# Autodesk Inventor assembly: chassis
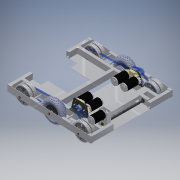
[picture p0: Inventor's stored thumbnail of the model, 180x180]
Saved by Autodesk Inventor 2016 (Build 200138000, 138)
## iProperties
Created: 2016-01-16
Part Number: chassis
Document SubType Name: Assembly
Designer: gus
Mass: 18782.9 g
Surface Area: 40799.8 cm^2
Volume: 7776.64 cm^3
Density: 2.4153 g/cm^3
Author: gus
## Documents named in this file (24)
- \\Mac\Home\Desktop\1510-stronghold-CAD-master\chassis\chassis.iam
- \\Mac\Home\Desktop\1510-stronghold-CAD-master\chassis\1x2x28.ipt
- \\Mac\Home\Desktop\1510-stronghold-CAD-master\chassis\1x2x19.ipt
- \\Mac\Home\Desktop\1510-stronghold-CAD-master\chassis\1x2x8in.ipt
- \\Mac\Home\Desktop\1510-stronghold-CAD-master\chassis\3 in churro.ipt
- \\Mac\Home\Desktop\1510-stronghold-CAD-master\chassis\side plate.ipt
- \\Mac\Home\Desktop\1510-stronghold-CAD-master\chassis\PneumaticWheel_am-0970-2.iam
- \\Mac\Home\Desktop\1510-stronghold-CAD-master\chassis\CIMple Box\CIMple Box.iam
- \\Mac\Home\Desktop\1510-stronghold-CAD-master\chassis\am-0736_S35-12DHE.ipt
- \\Mac\Home\Desktop\1510-stronghold-CAD-master\chassis\am-940a-6-HiGrip-.iam
- \\Mac\Home\Desktop\1510-stronghold-CAD-master\chassis\half-inch hex bolt.ipt
- \\Mac\Home\Desktop\1510-stronghold-CAD-master\chassis\half-inch hex nut.ipt
- \\Mac\Home\Desktop\1510-stronghold-CAD-master\chassis\wheel arm support.ipt
- \\Mac\Home\Desktop\1510-stronghold-CAD-master\roller wheels\toughbox micro\Toughbox+Nano+All+Shafts+v2-2.iam
- \\Mac\Home\Desktop\1510-stronghold-CAD-master\roller wheels\hex bearing.ipt
- \\Mac\Home\Desktop\1510-stronghold-CAD-master\chassis\chassis\Design Accelerator\Chain Drive13.iam
- \\Mac\Home\Desktop\1510-stronghold-CAD-master\chassis\chassis\Design Accelerator\Chain Drive14.iam
- \\Mac\Home\Desktop\1510-stronghold-CAD-master\chassis\chassis\Design Accelerator\Chain Drive15.iam
- \\Mac\Home\Desktop\1510-stronghold-CAD-master\chassis\chassis\Design Accelerator\Chain Drive16.iam
- \\Mac\Home\Desktop\1510-stronghold-CAD-master\chassis\chassis\Design Accelerator\Chain Drive17.iam
- \\Mac\Home\Desktop\1510-stronghold-CAD-master\chassis\skid plate.ipt
- \\Mac\Home\Desktop\1510-stronghold-CAD-master\chassis\request-piano-hinge-1\PIANO HINGE.iam
- \\Mac\Home\Desktop\1510-stronghold-CAD-master\chassis\skid plate back.ipt
- \\Mac\Home\Desktop\1510-stronghold-CAD-master\chassis\skid strip.ipt
## Components (52 placed, 19 different names)
1. 1x2x28:1 — Mate:1, Mate:2, Flush:2, Mate:4, Flush:4, Flush:6, Mate:19, Rotational:7, Rotational:8, Cylindrical:25, Rotational:18, Rotational:29, Cylindrical:22, Mate:41, Mate:57, Mate:58, Flush:49, Flush:53
2. 1x2x19:1 — Mate:1, Flush:2, Mate:12, Mate:13, Flush:22
3. 1x2x19:2 — Mate:2, Mate:34, Flush:43, Flush:44, Mate:71, Mate:72, Flush:48, Mate:73
4. 1x2x8in:1 — Mate:8, Flush:10, Mate:13, Mate:35, Flush:52
5. 1x2x8in:2 — Mate:4, Flush:4, Flush:6, Mate:9, Flush:11, Mate:12, Mate:62
6. 3 in churro:1 — Mate:10, Mate:67
7. 3 in churro:2 — Mate:11, Mate:65
8. 3 in churro:3 — Mate:36, Mate:69
9. 3 in churro:4 — Mate:37, Mate:70
10. side plate:1 — Mate:8, Flush:10, Mate:21, Rotational:23, Rotational:24, Rotational:25, Mate:61, Mate:63, Mate:68, Mate:69, Mate:70
11. side plate:2 — Mate:9, Flush:11, Mate:10, Mate:11, Mate:22, Rotational:26, Rotational:27, Rotational:28, Mate:62, Mate:64, Mate:65, Mate:66, Mate:67, Mate:77
12. PneumaticWheel_am-0970-2:1 [sub-assembly] — Rotational:20, Flush:39, Flush:40
13. 1x2x8in:3 — Mate:19, Mate:22, Mate:53, Flush:34, Flush:54, Mate:77, Flush:56
14. 1x2x8in:4 — Mate:21, Mate:33, Flush:20, Flush:21, Flush:28, Mate:39, Mate:61, Flush:56, Flush:57
15. am-0736_S35-12DHE:1 — Cylindrical:2, Mate:49
16. am-0736_S35-12DHE:2 — Mate:50, Cylindrical:26
17. am-940a-6-HiGrip-:1 [sub-assembly] — Cylindrical:25, Flush:42
18. am-940a-6-HiGrip-:2 [sub-assembly] — Cylindrical:22, Flush:41
19. am-940a-6-HiGrip-:3 [sub-assembly] — Cylindrical:23, Flush:40
20. am-940a-6-HiGrip-:4 [sub-assembly] — Cylindrical:24, Flush:39
21. half-inch hex bolt:2 — Rotational:12
22. half-inch hex bolt:4 — Rotational:14
23. half-inch hex bolt:5 — Rotational:7
24. half-inch hex bolt:6 — Rotational:8
25. PneumaticWheel_am-0970-2:2 [sub-assembly] — Rotational:29, Flush:41, Flush:42
26. 1x2x28:2 — Mate:33, Flush:20, Mate:34, Flush:21, Mate:35, Flush:22, Mate:36, Mate:37, Rotational:12, Rotational:14, Cylindrical:24, Rotational:17, Rotational:20, Cylindrical:23, Mate:42, Mate:55, Mate:56, Flush:43, Flush:47, Mate:75, Flush:55, Mate:79
27. half-inch hex bolt:7 — Rotational:17
28. half-inch hex bolt:8 — Rotational:18
29. half-inch hex nut:1 — Rotational:23
30. half-inch hex nut:2 — Rotational:27
31. half-inch hex nut:3 — Rotational:25
32. half-inch hex nut:4 — Rotational:26
33. half-inch hex nut:5 — Rotational:28
34. half-inch hex nut:6 — Rotational:24
35. wheel arm support:1 — Flush:28, Mate:39, Rotational:30, Flush:44, Mate:71
36. CIMple Box:1 [sub-assembly] — Mate:41, Mate:50, Cylindrical:26, Flush:49, Mate:73
37. CIMple Box:2 [sub-assembly] — Mate:42, Cylindrical:2, Mate:49, Flush:47, Flush:48
38. Toughbox+Nano+All+Shafts+v2-2:1 [sub-assembly] — Mate:53, Flush:34, Mate:54, Mate:72
39. hex bearing:1 — Rotational:30, Mate:54
40. 3 in churro:5 — Mate:55, Mate:63
41. 3 in churro:6 — Mate:56, Mate:68
42. 3 in churro:7 — Mate:57, Mate:64
43. 3 in churro:8 — Mate:58, Mate:66
44. Chain Drive:1 [sub-assembly]
45. Chain Drive:2 [sub-assembly]
46. Chain Drive:3 [sub-assembly]
47. Chain Drive:4 [sub-assembly]
48. Chain Drive:5 [sub-assembly]
49. skid plate:2 — Mate:75, Flush:52
50. PIANO HINGE:1 [sub-assembly] — Mate:78, Mate:79, Flush:58, Flush:59, Mate:80
51. skid plate back:1 — Flush:53, Flush:59, Mate:80
52. skid strip:1 — Flush:54, Flush:55, Flush:57, Mate:78, Flush:58
## Relationships (94: Mate 46, Flush 27, RevoluteJoint 15, CylindricalJoint 6)
- Mate:1: 1x2x28:1 ↔ 1x2x19:1
- Mate:2: 1x2x28:1 ↔ 1x2x19:2
- Flush:2: 1x2x28:1 ↔ 1x2x19:1
- Mate:4: 1x2x28:1 ↔ 1x2x8in:2
- Flush:4: 1x2x28:1 ↔ 1x2x8in:2
- Flush:6 (101.6 mm): 1x2x28:1 ↔ 1x2x8in:2
- Mate:8: 1x2x8in:1 ↔ side plate:1
- Mate:9: 1x2x8in:2 ↔ side plate:2
- Flush:10: 1x2x8in:1 ↔ side plate:1
- Flush:11: 1x2x8in:2 ↔ side plate:2
- Mate:10: 3 in churro:1 ↔ side plate:2
- Mate:11: 3 in churro:2 ↔ side plate:2
- Mate:12 (304.8 mm): 1x2x19:1 ↔ 1x2x8in:2
- Mate:13 (304.8 mm): 1x2x19:1 ↔ 1x2x8in:1
- Mate:19: 1x2x28:1 ↔ 1x2x8in:3
- Mate:21: side plate:1 ↔ 1x2x8in:4
- Mate:22: side plate:2 ↔ 1x2x8in:3
- Rotational:7 [RevoluteJoint]: 1x2x28:1 ↔ half-inch hex bolt:5
- Rotational:8 [RevoluteJoint]: 1x2x28:1 ↔ half-inch hex bolt:6
- Mate:33: 1x2x8in:4 ↔ 1x2x28:2
- Flush:20: 1x2x8in:4 ↔ 1x2x28:2
- Mate:34: 1x2x19:2 ↔ 1x2x28:2
- Flush:21 (101.6 mm): 1x2x8in:4 ↔ 1x2x28:2
- Mate:35: 1x2x8in:1 ↔ 1x2x28:2
- Flush:22: 1x2x19:1 ↔ 1x2x28:2
- Mate:36: 3 in churro:3 ↔ 1x2x28:2
- Mate:37: 3 in churro:4 ↔ 1x2x28:2
- Rotational:12 [RevoluteJoint]: half-inch hex bolt:2 ↔ 1x2x28:2
- Rotational:14 [RevoluteJoint]: half-inch hex bolt:4 ↔ 1x2x28:2
- Cylindrical:22: 1x2x28:1 ↔ am-940a-6-HiGrip-:2
- Cylindrical:24: am-940a-6-HiGrip-:4 ↔ 1x2x28:2
- Cylindrical:23: am-940a-6-HiGrip-:3 ↔ 1x2x28:2
- Cylindrical:25: 1x2x28:1 ↔ am-940a-6-HiGrip-:1
- Rotational:17 [RevoluteJoint]: 1x2x28:2 ↔ half-inch hex bolt:7
- Rotational:18 [RevoluteJoint]: 1x2x28:1 ↔ half-inch hex bolt:8
- Rotational:20 [RevoluteJoint]: PneumaticWheel_am-0970-2:1 ↔ 1x2x28:2
- Rotational:29 [RevoluteJoint]: 1x2x28:1 ↔ PneumaticWheel_am-0970-2:2
- Rotational:23 [RevoluteJoint]: side plate:1 ↔ half-inch hex nut:1
- Rotational:24 [RevoluteJoint]: side plate:1 ↔ half-inch hex nut:6
- Rotational:25 [RevoluteJoint]: side plate:1 ↔ half-inch hex nut:3
- Rotational:26 [RevoluteJoint]: side plate:2 ↔ half-inch hex nut:4
- Rotational:27 [RevoluteJoint]: side plate:2 ↔ half-inch hex nut:2
- Rotational:28 [RevoluteJoint]: side plate:2 ↔ half-inch hex nut:5
- Flush:28: 1x2x8in:4 ↔ wheel arm support:1
- Mate:39: 1x2x8in:4 ↔ wheel arm support:1
- Mate:41: 1x2x28:1 ↔ CIMple Box:1
- Mate:42: 1x2x28:2 ↔ CIMple Box:2
- Cylindrical:2: am-0736_S35-12DHE:1 ↔ CIMple Box:2
- Mate:49: am-0736_S35-12DHE:1 ↔ CIMple Box:2
- Mate:50: am-0736_S35-12DHE:2 ↔ CIMple Box:1
- Cylindrical:26: am-0736_S35-12DHE:2 ↔ CIMple Box:1
- Mate:53: 1x2x8in:3 ↔ Toughbox+Nano+All+Shafts+v2-2:1
- Flush:34: 1x2x8in:3 ↔ Toughbox+Nano+All+Shafts+v2-2:1
- Rotational:30 [RevoluteJoint]: wheel arm support:1 ↔ hex bearing:1
- Mate:54: Toughbox+Nano+All+Shafts+v2-2:1 ↔ hex bearing:1
- Mate:55: 1x2x28:2 ↔ 3 in churro:5
- Mate:56: 1x2x28:2 ↔ 3 in churro:6
- Mate:57: 1x2x28:1 ↔ 3 in churro:7
- Mate:58: 1x2x28:1 ↔ 3 in churro:8
- Flush:39: PneumaticWheel_am-0970-2:1 ↔ am-940a-6-HiGrip-:4
- Flush:40: PneumaticWheel_am-0970-2:1 ↔ am-940a-6-HiGrip-:3
- Flush:41: am-940a-6-HiGrip-:2 ↔ PneumaticWheel_am-0970-2:2
- Flush:42: am-940a-6-HiGrip-:1 ↔ PneumaticWheel_am-0970-2:2
- Mate:61: side plate:1 ↔ 1x2x8in:4
- Mate:62: 1x2x8in:2 ↔ side plate:2
- Mate:63: side plate:1 ↔ 3 in churro:5
- Mate:64: side plate:2 ↔ 3 in churro:7
- Mate:65: 3 in churro:2 ↔ side plate:2
- Mate:66: side plate:2 ↔ 3 in churro:8
- Mate:67: 3 in churro:1 ↔ side plate:2
- Mate:68: side plate:1 ↔ 3 in churro:6
- Mate:69: 3 in churro:3 ↔ side plate:1
- Mate:70: 3 in churro:4 ↔ side plate:1
- Flush:43: 1x2x19:2 ↔ 1x2x28:2
- Flush:44 (10.0076 mm): 1x2x19:2 ↔ wheel arm support:1
- Mate:71: 1x2x19:2 ↔ wheel arm support:1
- Mate:72: 1x2x19:2 ↔ Toughbox+Nano+All+Shafts+v2-2:1
- Flush:47: 1x2x28:2 ↔ CIMple Box:2
- Flush:48 (50.8 mm): 1x2x19:2 ↔ CIMple Box:2
- Flush:49: 1x2x28:1 ↔ CIMple Box:1
- Mate:73: 1x2x19:2 ↔ CIMple Box:1
- Mate:75: 1x2x28:2 ↔ skid plate:2
- Flush:52: 1x2x8in:1 ↔ skid plate:2
- Flush:53: 1x2x28:1 ↔ skid plate back:1
- Flush:54: 1x2x8in:3 ↔ skid strip:1
- Flush:55: 1x2x28:2 ↔ skid strip:1
- Mate:77: side plate:2 ↔ 1x2x8in:3
- Flush:56: 1x2x8in:3 ↔ 1x2x8in:4
- Flush:57: 1x2x8in:4 ↔ skid strip:1
- Mate:78: PIANO HINGE:1 ↔ skid strip:1
- Mate:79 (88.9 mm): 1x2x28:2 ↔ PIANO HINGE:1
- Flush:58: PIANO HINGE:1 ↔ skid strip:1
- Flush:59: PIANO HINGE:1 ↔ skid plate back:1
- Mate:80: PIANO HINGE:1 ↔ skid plate back:1
